# Autodesk Inventor assembly: RS-550_Assembly
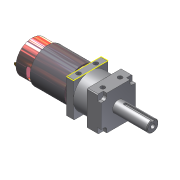
[picture p0: Inventor's stored thumbnail of the model, 180x180]
Saved by Autodesk Inventor 2012 (Build 160160000, 160)
## iProperties
Created: 2012-02-21
Part Number: RS-550_Assembly
Document SubType Name: Assembly
Designer: JesseK
Author: JesseK
## Documents named in this file (3)
- Z:\UserData\Documents\Inventor\team1885frc\Banebots\RS-550_Assembly.iam
- Z:\UserData\Documents\Inventor\team1885frc\Banebots\P60Gearbox_1stage.ipt
- Z:\UserData\Documents\Inventor\team1885frc\Banebots\BaneBots_RS-550.ipt
## Components (2 placed, 2 different names)
1. P60Gearbox_1stage:1 — Mate:1, Mate:2
2. BaneBots_RS-550:1 — Mate:1, Mate:2
## Relationships (2: Mate 2)
- Mate:1: P60Gearbox_1stage:1 ↔ BaneBots_RS-550:1
- Mate:2: P60Gearbox_1stage:1 ↔ BaneBots_RS-550:1
